# Autodesk Inventor assembly: Inner Gear
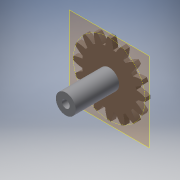
[picture p0: Inventor's stored thumbnail of the model, 180x180]
Saved by Autodesk Inventor 2016 (Build 200138000, 138)
## iProperties
Created: 2016-04-25
Part Number: Inner Gear
Document SubType Name: Assembly
Designer: rubenjm
Author: rubenjm
## Documents named in this file (3)
- C:\Users\rubenjm\Documents\To Transfer\2k16 Spring\RME\GGC\V3\Inner Gear.iam
- C:\Users\rubenjm\Documents\To Transfer\2k16 Spring\RME\GGC\V3\Turntable Outer Gear\Design Accelerator\Spur Gear12.ipt
- C:\Users\rubenjm\Documents\To Transfer\2k16 Spring\RME\GGC\V3\Inner Gear Extruded.ipt
## Components (2 placed, 2 different names)
1. Spur Gear1:1 — Flush:1, Flush:2
2. Inner Gear Extruded:1 — Flush:1, Flush:2
## Relationships (2: Flush 2)
- Flush:1: Spur Gear1:1 ↔ Inner Gear Extruded:1
- Flush:2: Spur Gear1:1 ↔ Inner Gear Extruded:1
